# Autodesk Inventor assembly: Assembly3,1
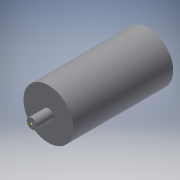
[picture p0: Inventor's stored thumbnail of the model, 180x180]
Saved by Autodesk Inventor 2019 (Build 230136000, 136)
## iProperties
Created: 2021-08-31
Part Number: Assembly3,1
Material: 一般
Document SubType Name: Assembly
Designer: yuta
Author: yuta
## Documents named in this file (3)
- C:\Users\yuta\Documents\キャチロボ\Assembly3,1.iam
- C:\Users\yuta\Documents\キャチロボ\Part23.ipt
- C:\Users\yuta\Documents\キャチロボ\Part24.ipt
## Components (2 placed, 2 different names)
1. Part23:1 — メイト:1, メイト:2
2. Part24:1 — メイト:1, メイト:2
## Relationships (2: Mate 2)
- メイト:1 [Mate]: Part23:1 ↔ Part24:1
- メイト:2 [Mate]: Part23:1 ↔ Part24:1
